# Autodesk Inventor assembly: Lathe Model V3
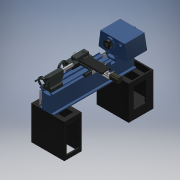
[picture p0: Inventor's stored thumbnail of the model, 180x180]
Saved by Autodesk Inventor 2018 (Build 220112000, 112)
## iProperties
Created: 2017-05-02
Part Number: Lathe Model V3
Document SubType Name: Assembly
Designer: M228544
Author: M228544
## Documents named in this file (31)
- E:\Miguel\Miguel 1\Miguel\Lathe with updated parts (LATEST of 20 06 17)\Lathe Model V3.iam
- E:\Miguel\Miguel 1\Miguel\Lathe with updated parts (LATEST of 20 06 17)\BED.ipt
- E:\Miguel\Miguel 1\Miguel\Lathe with updated parts (LATEST of 20 06 17)\saddle.ipt
- E:\Miguel\Miguel 1\Miguel\Lathe with updated parts (LATEST of 20 06 17)\Bottom-Tool-Bit.ipt
- E:\Miguel\Miguel 1\Miguel\Lathe with updated parts (LATEST of 20 06 17)\Top-Part-Tool-bit.ipt
- E:\Miguel\Miguel 1\Miguel\Lathe with updated parts (LATEST of 20 06 17)\tail stock - body part.ipt
- E:\Miguel\Miguel 1\Miguel\Lathe with updated parts (LATEST of 20 06 17)\Gearbox.ipt
- E:\Miguel\Miguel 1\Miguel\Lathe with updated parts (LATEST of 20 06 17)\Left leg.ipt
- E:\Miguel\Miguel 1\Miguel\Lathe with updated parts (LATEST of 20 06 17)\Right Leg.ipt
- E:\Miguel\Miguel 1\Miguel\Lathe with updated parts (LATEST of 20 06 17)\Apron.ipt
- E:\Miguel\Miguel 1\Miguel\Lathe with updated parts (LATEST of 20 06 17)\AIS2016\BNT 2010-2_6 +1166L C7T-J1K_10000KBK 15BF 15.iam
- E:\Miguel\Miguel 1\Miguel\Lathe with updated parts (LATEST of 20 06 17)\Servo Motor\Servo Motor.iam
- E:\Miguel\Miguel 1\Miguel\Lathe with updated parts (LATEST of 20 06 17)\Ball screw nut and apron join.ipt
- E:\Miguel\Miguel 1\Miguel\Lathe with updated parts (LATEST of 20 06 17)\barrel.ipt
- E:\Miguel\Miguel 1\Miguel\Lathe with updated parts (LATEST of 20 06 17)\connecting wheel.ipt
- E:\Miguel\Miguel 1\Miguel\Lathe with updated parts (LATEST of 20 06 17)\chuck holder.ipt
- E:\Miguel\Miguel 1\Miguel\Lathe with updated parts (LATEST of 20 06 17)\Chuck shaft.ipt
- E:\Miguel\Miguel 1\Miguel\Lathe with updated parts (LATEST of 20 06 17)\MotorHolderLongAxis.ipt
- E:\Miguel\Miguel 1\Miguel\Lathe with updated parts (LATEST of 20 06 17)\MotorHolderLongAxisTop.ipt
- E:\Miguel\Miguel 1\Miguel\Lathe with updated parts (LATEST of 20 06 17)\MotorHolderLongAxisBottom.ipt
- E:\Miguel\Miguel 1\Miguel\Lathe with updated parts (LATEST of 20 06 17)\DriveSideBallScrewSupport.ipt
- E:\Miguel\Miguel 1\Miguel\Lathe with updated parts (LATEST of 20 06 17)\DrivenSideBallScrewSupport.ipt
- E:\with new modification of the X axis - last version\slide-ontop-of-saddle(fixed).ipt
- E:\with new modification of the X axis - last version\BaseSupport X axis-UcTran\BaseSupport.ipt
- E:\with new modification of the X axis - last version\X Axis Nut Correct\Rosses spaces and ball screw bearing.iam
- E:\with new modification of the X axis - last version\BaseSupport X axis-UcTran\X-Axis.ipt
- E:\with new modification of the X axis - last version\block for gear x-axis.ipt
- E:\with new modification of the X axis - last version\short shaft x axis\608ZZ Ball Screw Support Unit.ipt
- E:\with new modification of the X axis - last version\flexible coupling X axis.ipt
- E:\with new modification of the X axis - last version\X Axis Nut Correct\Nut Bracket.ipt
- E:\with new modification of the X axis - last version\X Axis Nut Correct\Correct nut assembly (modified).iam
## Components (32 placed, 31 different names)
1. BED:1 — Mate:1, Mate:2, Mate:9, Mate:10, Mate:11, Flush:5, Flush:6, Mate:13, Mate:14, Flush:7, Flush:9, Mate:58, Angle:7, Mate:59, Mate:63, Angle:8, Mate:64, Flush:38
2. saddle:1 — Mate:1, Mate:2, Flush:10, Flush:11, Mate:15, Mate:20, Mate:75, Mate:76, Flush:40, Mate:80, Mate:81, Angle:12, Mate:82, Angle:13, Mate:83
3. Bottom-Tool-Bit:1 — Mate:3, Mate:4, Flush:14
4. Top-Part-Tool-bit:1 — Mate:3, Mate:4, Flush:14, Mate:78, Angle:11, Mate:79
5. tail stock - body part:1 — Mate:9, Mate:10, Flush:13, Mate:19, Mate:20, Mate:35, Mate:38, Flush:33
6. Gearbox:1 — Mate:11, Flush:5, Flush:13, Mate:19, Mate:21, Mate:39, Mate:40
7. Left leg:1 — Mate:14, Flush:7, Flush:8
8. Right Leg:1 — Flush:6, Mate:13, Flush:8, Flush:9
9. Apron:1 — Flush:10, Flush:11, Mate:15, Mate:21, Angle:10, Flush:41, Mate:103, Angle:15, Flush:42
10. BNT 2010-2_6 +1166L C7T-J1K_10000KBK 15BF 15:1 [sub-assembly] — Mate:60, Mate:61, Mate:62, Flush:38, Mate:66, Mate:69, Mate:102, Angle:15, Flush:42, Flush:43
11. Servo Motor:1 [sub-assembly] — Mate:67, Mate:68, Angle:9, Mate:69, Mate:101
12. Ball screw nut and apron join:1 — Flush:41, Mate:103, Flush:43
13. barrel:1 — Mate:35, Mate:36, Mate:37, Rotation/Translation:1, Flush:33
14. connecting wheel:1 — Mate:36, Mate:37, Mate:38, Rotation/Translation:1
15. chuck holder:1 — Mate:39, Mate:40, Mate:41, Mate:42
16. Chuck shaft:1 — Mate:41, Mate:42
17. MotorHolderLongAxisTop:1 — Mate:70, Flush:39, Mate:71
18. MotorHolderLongAxisBottom:1 — Mate:72, Mate:73, Mate:74
19. DriveSideBallScrewSupport:1 — Mate:58, Angle:7, Mate:59, Mate:60, Mate:61, Mate:62, Mate:65, Flush:39, Mate:71, Mate:72
20. DrivenSideBallScrewSupport:1 — Mate:63, Angle:8, Mate:64
21. MotorHolderLongAxis:1 — Mate:65, Mate:66, Mate:67, Mate:68, Angle:9, Mate:70, Mate:73, Mate:74
22. slide-ontop-of-saddle(fixed):1 — Mate:75, Angle:10, Mate:76, Flush:40, Mate:78, Angle:11, Mate:79, Mate:96, Mate:97, Mate:98
23. BaseSupport:1 — Mate:80, Mate:81, Angle:12, Mate:84, Mate:85, Mate:86, Mate:89, Mate:90, Mate:91
24. Rosses spaces and ball screw bearing:1 [sub-assembly] — Mate:82, Angle:13, Mate:83
25. Servo Motor:2 [sub-assembly] — Mate:84, Mate:85, Mate:86, Mate:87, Mate:88, Mate:94, Mate:95
26. X-Axis:1 — Mate:87, Mate:88, Mate:99
27. block for gear x-axis:1 — Mate:89, Mate:90, Mate:91, Mate:92, Mate:93
28. 608ZZ Ball Screw Support Unit:1 — Mate:92, Mate:93
29. flexible coupling X axis:1 — Mate:94, Mate:95
30. Nut Bracket:1 — Mate:96, Mate:97, Mate:98, Mate:100, Angle:14
31. Correct nut assembly (modified):1 [sub-assembly] — Mate:99, Mate:100, Angle:14
32. flexible coupling y axis:2 — Mate:101, Mate:102
## Relationships (92: Mate 66, Flush 16, Angle 9, RelateRotateTranslate 1)
- Mate:1: BED:1 ↔ saddle:1
- Mate:2: BED:1 ↔ saddle:1
- Mate:3: Bottom-Tool-Bit:1 ↔ Top-Part-Tool-bit:1
- Mate:4: Bottom-Tool-Bit:1 ↔ Top-Part-Tool-bit:1
- Mate:9: BED:1 ↔ tail stock - body part:1
- Mate:10: BED:1 ↔ tail stock - body part:1
- Mate:11: BED:1 ↔ Gearbox:1
- Flush:5: BED:1 ↔ Gearbox:1
- Flush:13: tail stock - body part:1 ↔ Gearbox:1
- Flush:6: BED:1 ↔ Right Leg:1
- Mate:13: BED:1 ↔ Right Leg:1
- Mate:14: BED:1 ↔ Left leg:1
- Flush:7: BED:1 ↔ Left leg:1
- Flush:8: Left leg:1 ↔ Right Leg:1
- Flush:9 (145 mm): BED:1 ↔ Right Leg:1
- Flush:10: saddle:1 ↔ Apron:1
- Flush:11: saddle:1 ↔ Apron:1
- Mate:15: saddle:1 ↔ Apron:1
- Flush:14: Bottom-Tool-Bit:1 ↔ Top-Part-Tool-bit:1
- Mate:19: tail stock - body part:1 ↔ Gearbox:1
- Mate:20: saddle:1 ↔ tail stock - body part:1
- Mate:21: Gearbox:1 ↔ Apron:1
- Mate:35: tail stock - body part:1 ↔ barrel:1
- Mate:36: barrel:1 ↔ connecting wheel:1
- Mate:37: barrel:1 ↔ connecting wheel:1
- Mate:38: tail stock - body part:1 ↔ connecting wheel:1
- Rotation/Translation:1 [RelateRotateTranslate] (100 mm): barrel:1 ↔ connecting wheel:1
- Flush:33: tail stock - body part:1 ↔ barrel:1
- Mate:39: Gearbox:1 ↔ chuck holder:1
- Mate:40 (0.46 mm): Gearbox:1 ↔ chuck holder:1
- Mate:41: chuck holder:1 ↔ Chuck shaft:1
- Mate:42 (11.2 mm): chuck holder:1 ↔ Chuck shaft:1
- Mate:58: BED:1 ↔ DriveSideBallScrewSupport:1
- Angle:7 (0 deg): BED:1 ↔ DriveSideBallScrewSupport:1
- Mate:59: BED:1 ↔ DriveSideBallScrewSupport:1
- Mate:60: BNT 2010-2_6 +1166L C7T-J1K_10000KBK 15BF 15:1 ↔ DriveSideBallScrewSupport:1
- Mate:61: BNT 2010-2_6 +1166L C7T-J1K_10000KBK 15BF 15:1 ↔ DriveSideBallScrewSupport:1
- Mate:62: BNT 2010-2_6 +1166L C7T-J1K_10000KBK 15BF 15:1 ↔ DriveSideBallScrewSupport:1
- Mate:63: BED:1 ↔ DrivenSideBallScrewSupport:1
- Angle:8 (0 deg): BED:1 ↔ DrivenSideBallScrewSupport:1
- Mate:64: BED:1 ↔ DrivenSideBallScrewSupport:1
- Flush:38 (10 mm): BED:1 ↔ BNT 2010-2_6 +1166L C7T-J1K_10000KBK 15BF 15:1
- Mate:65: DriveSideBallScrewSupport:1 ↔ MotorHolderLongAxis:1
- Mate:66: BNT 2010-2_6 +1166L C7T-J1K_10000KBK 15BF 15:1 ↔ MotorHolderLongAxis:1
- Mate:67: Servo Motor:1 ↔ MotorHolderLongAxis:1
- Mate:68: Servo Motor:1 ↔ MotorHolderLongAxis:1
- Angle:9 (45 deg): Servo Motor:1 ↔ MotorHolderLongAxis:1
- Mate:69 (20 mm): BNT 2010-2_6 +1166L C7T-J1K_10000KBK 15BF 15:1 ↔ Servo Motor:1
- Mate:70: MotorHolderLongAxisTop:1 ↔ MotorHolderLongAxis:1
- Flush:39 (40 mm): MotorHolderLongAxisTop:1 ↔ DriveSideBallScrewSupport:1
- Mate:71: MotorHolderLongAxisTop:1 ↔ DriveSideBallScrewSupport:1
- Mate:72: MotorHolderLongAxisBottom:1 ↔ DriveSideBallScrewSupport:1
- Mate:73: MotorHolderLongAxisBottom:1 ↔ MotorHolderLongAxis:1
- Mate:74: MotorHolderLongAxisBottom:1 ↔ MotorHolderLongAxis:1
- Mate:75: saddle:1 ↔ slide-ontop-of-saddle(fixed):1
- Angle:10 (0 deg): Apron:1 ↔ slide-ontop-of-saddle(fixed):1
- Mate:76: saddle:1 ↔ slide-ontop-of-saddle(fixed):1
- Flush:40: saddle:1 ↔ slide-ontop-of-saddle(fixed):1
- Mate:78: Top-Part-Tool-bit:1 ↔ slide-ontop-of-saddle(fixed):1
- Angle:11 (270 deg): Top-Part-Tool-bit:1 ↔ slide-ontop-of-saddle(fixed):1
- Mate:79: Top-Part-Tool-bit:1 ↔ slide-ontop-of-saddle(fixed):1
- Mate:80: saddle:1 ↔ BaseSupport:1
- Mate:81: saddle:1 ↔ BaseSupport:1
- Angle:12 (0 deg): saddle:1 ↔ BaseSupport:1
- Mate:82: saddle:1 ↔ Rosses spaces and ball screw bearing:1
- Angle:13 (0 deg): saddle:1 ↔ Rosses spaces and ball screw bearing:1
- Mate:83: saddle:1 ↔ Rosses spaces and ball screw bearing:1
- Mate:84: BaseSupport:1 ↔ Servo Motor:2
- Mate:85: BaseSupport:1 ↔ Servo Motor:2
- Mate:86: BaseSupport:1 ↔ Servo Motor:2
- Mate:87: Servo Motor:2 ↔ X-Axis:1
- Mate:88 (10 mm): Servo Motor:2 ↔ X-Axis:1
- Mate:89: BaseSupport:1 ↔ block for gear x-axis:1
- Mate:90: BaseSupport:1 ↔ block for gear x-axis:1
- Mate:91: BaseSupport:1 ↔ block for gear x-axis:1
- Mate:92: block for gear x-axis:1 ↔ 608ZZ Ball Screw Support Unit:1
- Mate:93: block for gear x-axis:1 ↔ 608ZZ Ball Screw Support Unit:1
- Mate:94: Servo Motor:2 ↔ flexible coupling X axis:1
- Mate:95 (-15 mm): Servo Motor:2 ↔ flexible coupling X axis:1
- Mate:96: slide-ontop-of-saddle(fixed):1 ↔ Nut Bracket:1
- Mate:97: slide-ontop-of-saddle(fixed):1 ↔ Nut Bracket:1
- Mate:98: slide-ontop-of-saddle(fixed):1 ↔ Nut Bracket:1
- Mate:99: X-Axis:1 ↔ Correct nut assembly (modified):1
- Mate:100: Nut Bracket:1 ↔ Correct nut assembly (modified):1
- Angle:14 (0 deg): Nut Bracket:1 ↔ Correct nut assembly (modified):1
- Mate:101: Servo Motor:1 ↔ flexible coupling y axis:2
- Mate:102 (-10 mm): BNT 2010-2_6 +1166L C7T-J1K_10000KBK 15BF 15:1 ↔ flexible coupling y axis:2
- Flush:41: Apron:1 ↔ Ball screw nut and apron join:1
- Mate:103: Apron:1 ↔ Ball screw nut and apron join:1
- Angle:15 (180 deg): Apron:1 ↔ BNT 2010-2_6 +1166L C7T-J1K_10000KBK 15BF 15:1
- Flush:42 (10 mm): Apron:1 ↔ BNT 2010-2_6 +1166L C7T-J1K_10000KBK 15BF 15:1
- Flush:43: BNT 2010-2_6 +1166L C7T-J1K_10000KBK 15BF 15:1 ↔ Ball screw nut and apron join:1
